# Autodesk Inventor assembly: Full_shaft
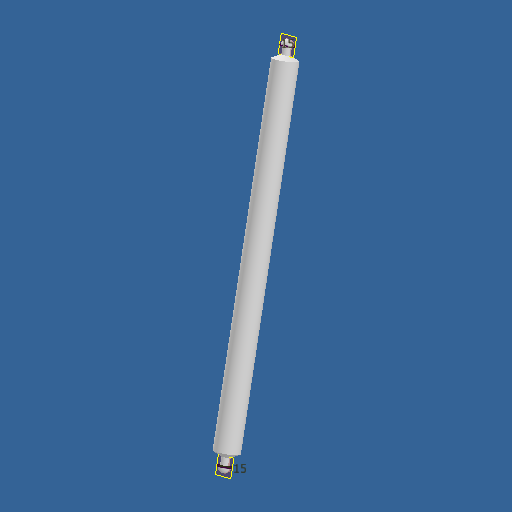
[picture p0: Inventor's stored thumbnail of the model, 512x512]
Saved by Autodesk Inventor 2026.2 (Build 302298000, 298)
## iProperties
Created: 2025-12-11
Part Number: Full_shaft
Document SubType Name: Assembly
Designer: Thoma
Author: Thoma
## Documents named in this file (2)
- C:\Users\Thoma\OneDrive\Desktop\dir\telescope_cover\telescope\version_3\Full_shaft.iam
- C:\Users\Thoma\OneDrive\Desktop\dir\telescope_cover\telescope\version_3\Shafts.ipt
## Components (2 placed, 1 different names)
1. Shafts:1 — Mate:1, Mate:2
2. Shafts:2 — Mate:1, Mate:2
## Relationships (2: Mate 2)
- Mate:1: Shafts:1 ↔ Shafts:2
- Mate:2: Shafts:1 ↔ Shafts:2
